# Autodesk Inventor assembly: derive_base_plate_v4
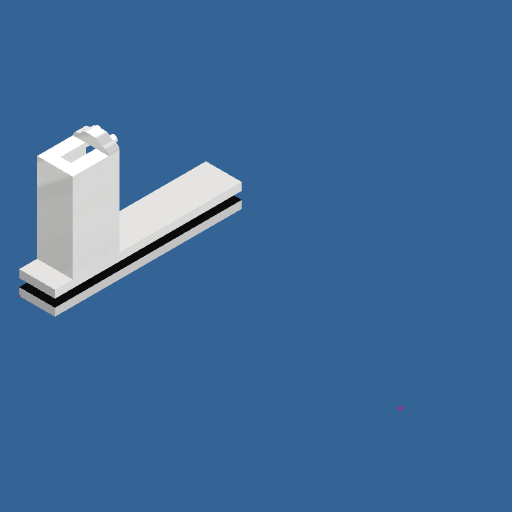
[picture p0: Inventor's stored thumbnail of the model, 512x512]
Saved by Autodesk Inventor 2026.2 (Build 302298000, 298)
## iProperties
Created: 2026-01-15
Part Number: derive_base_plate_v4
Document SubType Name: Assembly
Designer: Thoma
Author: Thoma
## Documents named in this file (3)
- C:\Users\Thoma\OneDrive\Desktop\dir\telescope_cover\cover\derive_base_plate_v4.iam
- C:\Users\Thoma\OneDrive\Desktop\dir\telescope_cover\cover\base+casing_v1.ipt
- C:\Users\Thoma\OneDrive\Desktop\dir\telescope_cover\cover\derive_Base_Plate_v3.ipt
## Components (2 placed, 2 different names)
1. base+casing_v1:1 — Mate:1, Flush:1, Flush:2
2. derive_Base_Plate_v3:1 — Mate:1, Flush:1, Flush:2
## Relationships (3: Flush 2, Mate 1)
- Mate:1 (5 mm): base+casing_v1:1 ↔ derive_Base_Plate_v3:1
- Flush:1: base+casing_v1:1 ↔ derive_Base_Plate_v3:1
- Flush:2: base+casing_v1:1 ↔ derive_Base_Plate_v3:1
